# Autodesk Inventor assembly: Rrwing cost
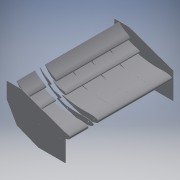
[picture p0: Inventor's stored thumbnail of the model, 180x180]
Saved by Autodesk Inventor 2018.3 (Build 223284000, 284)
## iProperties
Created: 2018-06-13
Part Number: Rrwing cost
Material: 一般
Document SubType Name: Assembly
Designer: ku_sk
Author: ku_sk
## Documents named in this file (5)
- D:\ku_sk\ドキュメント\Inventor\Aero\KS-15\コスト用CAD\Rrwing\Rrwing cost.iam
- D:\ku_sk\ドキュメント\Inventor\Aero\KS-15\コスト用CAD\Rrwing\parts\endplate.ipt
- D:\ku_sk\ドキュメント\Inventor\Aero\KS-15\コスト用CAD\Rrwing\parts\mainflap.ipt
- D:\ku_sk\ドキュメント\Inventor\Aero\KS-15\コスト用CAD\Rrwing\parts\splitter.ipt
- D:\ku_sk\ドキュメント\Inventor\Aero\KS-15\コスト用CAD\Rrwing\parts\subflap.ipt
## Components (21 placed, 4 different names)
1. endplate:1 — メイト:1, メイト:2, メイト:3, 角度:1, メイト:25, メイト:26, メイト:27
2. mainflap:1 — フラッシュ:1, メイト:2, メイト:3, メイト:4, メイト:5, メイト:6, メイト:10, メイト:11, メイト:12, フラッシュ:3
3. splitter:1 — メイト:10, メイト:11, メイト:12, メイト:13, メイト:14, メイト:15, メイト:21, メイト:22, メイト:46, メイト:47
4. subflap:1 — メイト:21, メイト:22, フラッシュ:3, フラッシュ:8
5. endplate:2 — メイト:37, メイト:38, メイト:39
6. mainflap:2 — メイト:13, メイト:14, メイト:15, メイト:16, メイト:17, メイト:18, フラッシュ:4
7. splitter:2 — メイト:16, メイト:17, メイト:18, メイト:23, メイト:24, メイト:28, メイト:29, メイト:34, メイト:40, メイト:41, メイト:48, メイト:49
8. subflap:2 — メイト:19, メイト:20, フラッシュ:2, フラッシュ:7
9. mainflap:3 — メイト:7, メイト:8, メイト:9, フラッシュ:2, メイト:25, メイト:26, メイト:27
10. splitter:3 — メイト:4, メイト:5, メイト:6, メイト:7, メイト:8, メイト:9, メイト:19, メイト:20, メイト:44, メイト:45
11. subflap:3 — メイト:23, メイト:24, フラッシュ:4, フラッシュ:9
12. mainflap:4 — メイト:28, メイト:29, メイト:30, メイト:31, メイト:32, メイト:33, メイト:34, メイト:35, フラッシュ:5
13. subflap:4 — メイト:40, メイト:41, フラッシュ:5, フラッシュ:10
14. mainflap:5 — メイト:30, メイト:31, メイト:36, メイト:37, メイト:38, メイト:39, フラッシュ:6, フラッシュ:11
15. subflap:5 — メイト:42, メイト:43, フラッシュ:6
16. splitter:4 — メイト:32, メイト:33, メイト:35, メイト:36, メイト:42, メイト:43, メイト:50, メイト:51, メイト:52, メイト:53
17. subflap:6 — メイト:44, メイト:45, フラッシュ:7
18. subflap:7 — メイト:46, メイト:47, フラッシュ:8
19. subflap:8 — メイト:48, メイト:49, フラッシュ:9
20. subflap:9 — メイト:50, メイト:51, フラッシュ:10
21. subflap:10 — メイト:52, メイト:53, フラッシュ:11
## Relationships (65: Mate 53, Flush 11, Angle 1)
- メイト:1 [Mate]: endplate:1
- フラッシュ:1 [Flush]: mainflap:1
- メイト:2 [Mate]: endplate:1 ↔ mainflap:1
- メイト:3 [Mate]: endplate:1 ↔ mainflap:1
- 角度:1 [Angle] (0 deg): endplate:1
- メイト:4 [Mate]: mainflap:1 ↔ splitter:3
- メイト:5 [Mate]: mainflap:1 ↔ splitter:3
- メイト:6 [Mate] (50 mm): mainflap:1 ↔ splitter:3
- メイト:7 [Mate] (50 mm): mainflap:3 ↔ splitter:3
- メイト:8 [Mate]: mainflap:3 ↔ splitter:3
- メイト:9 [Mate]: mainflap:3 ↔ splitter:3
- メイト:10 [Mate]: mainflap:1 ↔ splitter:1
- メイト:11 [Mate]: mainflap:1 ↔ splitter:1
- メイト:12 [Mate]: mainflap:1 ↔ splitter:1
- メイト:13 [Mate]: splitter:1 ↔ mainflap:2
- メイト:14 [Mate]: splitter:1 ↔ mainflap:2
- メイト:15 [Mate]: splitter:1 ↔ mainflap:2
- メイト:16 [Mate]: mainflap:2 ↔ splitter:2
- メイト:17 [Mate]: mainflap:2 ↔ splitter:2
- メイト:18 [Mate]: mainflap:2 ↔ splitter:2
- メイト:19 [Mate]: subflap:2 ↔ splitter:3
- メイト:20 [Mate]: subflap:2 ↔ splitter:3
- メイト:21 [Mate]: splitter:1 ↔ subflap:1
- メイト:22 [Mate]: splitter:1 ↔ subflap:1
- メイト:23 [Mate]: splitter:2 ↔ subflap:3
- メイト:24 [Mate]: splitter:2 ↔ subflap:3
- フラッシュ:2 [Flush]: subflap:2 ↔ mainflap:3
- フラッシュ:3 [Flush]: mainflap:1 ↔ subflap:1
- フラッシュ:4 [Flush]: mainflap:2 ↔ subflap:3
- メイト:25 [Mate]: endplate:1 ↔ mainflap:3
- メイト:26 [Mate]: endplate:1 ↔ mainflap:3
- メイト:27 [Mate] (50 mm): endplate:1 ↔ mainflap:3
- メイト:28 [Mate]: splitter:2 ↔ mainflap:4
- メイト:29 [Mate]: splitter:2 ↔ mainflap:4
- メイト:30 [Mate]: mainflap:4 ↔ mainflap:5
- メイト:31 [Mate]: mainflap:4 ↔ mainflap:5
- メイト:32 [Mate]: mainflap:4 ↔ splitter:4
- メイト:33 [Mate]: mainflap:4 ↔ splitter:4
- メイト:34 [Mate]: splitter:2 ↔ mainflap:4
- メイト:35 [Mate]: mainflap:4 ↔ splitter:4
- メイト:36 [Mate]: mainflap:5 ↔ splitter:4
- メイト:37 [Mate]: endplate:2 ↔ mainflap:5
- メイト:38 [Mate]: endplate:2 ↔ mainflap:5
- メイト:39 [Mate]: endplate:2 ↔ mainflap:5
- メイト:40 [Mate]: splitter:2 ↔ subflap:4
- メイト:41 [Mate]: splitter:2 ↔ subflap:4
- メイト:42 [Mate]: subflap:5 ↔ splitter:4
- メイト:43 [Mate]: subflap:5 ↔ splitter:4
- フラッシュ:5 [Flush]: mainflap:4 ↔ subflap:4
- フラッシュ:6 [Flush]: mainflap:5 ↔ subflap:5
- メイト:44 [Mate]: splitter:3 ↔ subflap:6
- メイト:45 [Mate]: splitter:3 ↔ subflap:6
- フラッシュ:7 [Flush]: subflap:2 ↔ subflap:6
- メイト:46 [Mate]: splitter:1 ↔ subflap:7
- メイト:47 [Mate]: splitter:1 ↔ subflap:7
- フラッシュ:8 [Flush]: subflap:1 ↔ subflap:7
- メイト:48 [Mate]: splitter:2 ↔ subflap:8
- メイト:49 [Mate]: splitter:2 ↔ subflap:8
- メイト:50 [Mate]: splitter:4 ↔ subflap:9
- メイト:51 [Mate]: splitter:4 ↔ subflap:9
- フラッシュ:9 [Flush]: subflap:3 ↔ subflap:8
- フラッシュ:10 [Flush]: subflap:4 ↔ subflap:9
- メイト:52 [Mate]: splitter:4 ↔ subflap:10
- メイト:53 [Mate]: splitter:4 ↔ subflap:10
- フラッシュ:11 [Flush]: mainflap:5 ↔ subflap:10
